# Autodesk Inventor assembly: am14u3LongWithSlideMechanism
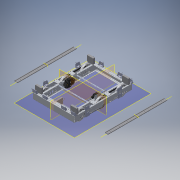
[picture p0: Inventor's stored thumbnail of the model, 180x180]
Saved by Autodesk Inventor 2018.2 (Build 222227000, 227)
## iProperties
Created: 2018-01-15
Part Number: am14u3LongWithSlideMechanism
Document SubType Name: Assembly
Designer: steele
Author: steele
## Documents named in this file (7)
- D:\snobotics\CAD-Development\robSteele\2018-FRC\am14u3LongWithSlideMechanism.iam
- D:\snobotics\CAD-Development\robSteele\2018-FRC\AMbaseLongWithBumper\Long with Bumper\DB_DriveBaseLong_AM14U3_Bumpers and Battery Tray.iam
- D:\snobotics\CAD-Development\robSteele\2018-FRC\Rail System\6109K422 rail 33 inches long.ipt
- D:\snobotics\CAD-Development\robSteele\2018-FRC\Rail System\supportBlock.ipt
- D:\snobotics\CAD-Development\robSteele\2018-FRC\Rail System\supportBlock_MIR.ipt
- D:\snobotics\CAD-Development\robSteele\2018-FRC\Rail System\supportBlock_MIR1.ipt
- D:\snobotics\CAD-Development\robSteele\2018-FRC\Rail System\supportBlock_MIR_MIR.ipt
## Components (7 placed, 6 different names)
1. DB_DriveBaseLong_AM14U3_Bumpers and Battery Tray:1 [sub-assembly] — Flush:2, Flush:3, Mate:1, Mate:2
2. 6109K422 rail 33 inches long:1
3. 6109K422 rail 33 inches long:2
4. supportBlock:1 — Flush:3, Mate:1, Mate:2
5. supportBlock_MIR:1
6. supportBlock_MIR1:1
7. supportBlock_MIR_MIR:1
## Relationships (4: Flush 2, Mate 2)
- Flush:2 (50.8 mm): DB_DriveBaseLong_AM14U3_Bumpers and Battery Tray:1
- Flush:3: DB_DriveBaseLong_AM14U3_Bumpers and Battery Tray:1 ↔ supportBlock:1
- Mate:1: DB_DriveBaseLong_AM14U3_Bumpers and Battery Tray:1 ↔ supportBlock:1
- Mate:2: DB_DriveBaseLong_AM14U3_Bumpers and Battery Tray:1 ↔ supportBlock:1
